# Autodesk Inventor assembly: Tracks Drag Chain Assembly
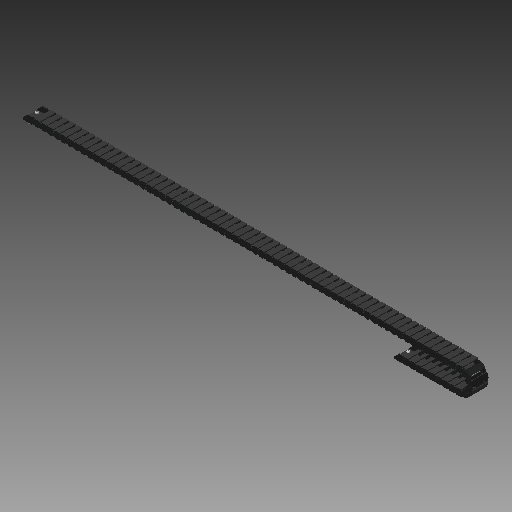
[picture p0: Inventor's stored thumbnail of the model, 512x512]
Saved by Autodesk Inventor 2017 (Build 210142000, 142)
## iProperties
Created: 2014-07-23
Part Number: Tracks Drag Chain Assembly
Document SubType Name: Assembly
Designer: umr
Sending System: SolidWorks 2014
Last Author: Rory
Last Saved: 2016-05-10
Author: umr
## Documents named in this file (7)
- C:\Users\Ali\Desktop\roboticFarm-master\Models2\CableCarier\Tracks Drag Chain Assembly.iam
- C:\Users\Ali\Desktop\roboticFarm-master\Original\SolidWorks 2014 Files\Drag Chain Link.ipt
- C:\Users\Ali\Desktop\roboticFarm-master\Original\SolidWorks 2014 Files\Drag Chain End 1.ipt
- C:\Users\Ali\Desktop\roboticFarm-master\Original\SolidWorks 2014 Files\Drag Chain End 2.ipt
- C:\Users\Ali\Desktop\roboticFarm-master\Models2\CableCarier\M5 Locknut.ipt
- C:\Users\Ali\Desktop\roboticFarm-master\Models2\CableCarier\M5 Screw_16mm.ipt
- C:\Users\Ali\Desktop\roboticFarm-master\Models2\CableCarier\M5 Washer.ipt
## Components (92 placed, 6 different names)
1. Drag Chain Link:208
2. Drag Chain Link:209
3. Drag Chain Link:210
4. Drag Chain Link:211
5. Drag Chain Link:212
6. Drag Chain Link:213
7. Drag Chain Link:214
8. Drag Chain Link:215
9. Drag Chain Link:216
10. Drag Chain Link:217
11. Drag Chain Link:218
12. Drag Chain Link:219
13. Drag Chain Link:220
14. Drag Chain Link:221
15. Drag Chain Link:222
16. Drag Chain Link:223
17. Drag Chain Link:224
18. Drag Chain Link:225
19. Drag Chain Link:226
20. Drag Chain Link:227
21. Drag Chain Link:228
22. Drag Chain Link:229
23. Drag Chain Link:230
24. Drag Chain Link:231
25. Drag Chain Link:232
26. Drag Chain Link:233
27. Drag Chain Link:234
28. Drag Chain Link:235
29. Drag Chain Link:236
30. Drag Chain Link:237
31. Drag Chain Link:238
32. Drag Chain Link:239
33. Drag Chain Link:240
34. Drag Chain Link:241
35. Drag Chain Link:242
36. Drag Chain Link:243
37. Drag Chain Link:244
38. Drag Chain Link:245
39. Drag Chain Link:246
40. Drag Chain Link:247
41. Drag Chain Link:248
42. Drag Chain Link:249
43. Drag Chain Link:250
44. Drag Chain Link:251
45. Drag Chain Link:252
46. Drag Chain Link:253
47. Drag Chain Link:254
48. Drag Chain Link:255
49. Drag Chain Link:256
50. Drag Chain Link:257
51. Drag Chain Link:258
52. Drag Chain Link:259
53. Drag Chain Link:260
54. Drag Chain Link:261
55. Drag Chain Link:262
56. Drag Chain Link:263
57. Drag Chain Link:264
58. Drag Chain Link:265
59. Drag Chain Link:266
60. Drag Chain Link:267
61. Drag Chain Link:268
62. Drag Chain Link:269
63. Drag Chain End 1:2 — Rigid:13, Rigid:14, Rigid:15, Rigid:16
64. Drag Chain End 2:2 — Rigid:9, Rigid:10, Rigid:11, Rigid:12
65. Drag Chain Link:270
66. Drag Chain Link:271
67. Drag Chain Link:272
68. Drag Chain Link:273
69. Drag Chain Link:274
70. Drag Chain Link:275
71. Drag Chain Link:276
72. Drag Chain Link:277
73. Drag Chain Link:278
74. Drag Chain Link:279
75. Drag Chain Link:280
76. Drag Chain Link:281
77. Drag Chain Link:282
78. Drag Chain Link:283
79. Drag Chain Link:284
80. Drag Chain Link:285
81. M5 Locknut:4 — Rigid:2
82. M5 Screw_16mm:4 — Rigid:15
83. M5 Washer:4 — Rigid:2, Rigid:16
84. M5 Locknut:5 — Rigid:7
85. M5 Screw_16mm:5 — Rigid:13
86. M5 Locknut:6 — Rigid:8
87. M5 Screw_16mm:6 — Rigid:11
88. M5 Locknut:7 — Rigid:6
89. M5 Screw_16mm:7 — Rigid:9
90. M5 Washer:5 — Rigid:7, Rigid:10
91. M5 Washer:6 — Rigid:6, Rigid:12
92. M5 Washer:7 — Rigid:8, Rigid:14
## Relationships (12: WeldJoint 12)
- Rigid:2 [WeldJoint]: M5 Locknut:4 ↔ M5 Washer:4
- Rigid:6 [WeldJoint]: M5 Locknut:7 ↔ M5 Washer:6
- Rigid:7 [WeldJoint]: M5 Locknut:5 ↔ M5 Washer:5
- Rigid:8 [WeldJoint]: M5 Locknut:6 ↔ M5 Washer:7
- Rigid:9 [WeldJoint]: Drag Chain End 2:2 ↔ M5 Screw_16mm:7
- Rigid:10 [WeldJoint]: Drag Chain End 2:2 ↔ M5 Washer:5
- Rigid:11 [WeldJoint]: Drag Chain End 2:2 ↔ M5 Screw_16mm:6
- Rigid:12 [WeldJoint]: Drag Chain End 2:2 ↔ M5 Washer:6
- Rigid:13 [WeldJoint]: Drag Chain End 1:2 ↔ M5 Screw_16mm:5
- Rigid:14 [WeldJoint]: Drag Chain End 1:2 ↔ M5 Washer:7
- Rigid:15 [WeldJoint]: Drag Chain End 1:2 ↔ M5 Screw_16mm:4
- Rigid:16 [WeldJoint]: Drag Chain End 1:2 ↔ M5 Washer:4
